# Autodesk Inventor assembly: ensemble
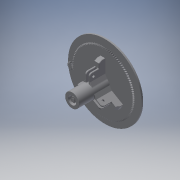
[picture p0: Inventor's stored thumbnail of the model, 180x180]
Saved by Autodesk Inventor 2019 (Build 230136000, 136)
## iProperties
Created: 2018-05-16
Part Number: ensemble
Material: Générique
Document SubType Name: Assembly
Designer: Theo
Author: Theo
## Documents named in this file (9)
- D:\dev\projects\canon-ace\ACE-T A\ensemble.iam
- D:\dev\projects\canon-ace\ACE-T A\support_principal.ipt
- D:\dev\projects\canon-ace\ACE-T A\axe_rotation_principal.ipt
- D:\dev\3d_parts\skf_6000\roulement_6000_2.iam
- D:\dev\3d_parts\emile_maurin_2201110\2201110.ipt
- D:\dev\projects\canon-ace\ACE-T A\engrenage_rotation.ipt
- D:\dev\projects\canon-ace\ACE-T A\tourelle.ipt
- D:\dev\projects\canon-ace\ACE-T A\support_serrage_tourelle.ipt
- D:\dev\projects\canon-ace\ACE-T A\engrenage_roation_1.ipt
## Components (9 placed, 8 different names)
1. support_principal:1 — Placage:1, Placage:2, Placage:4, Placage:5, Placage:6, Placage:9, Placage:10, Placage:11
2. axe_rotation_principal:1 — Placage:1, Placage:3, Placage:7, Logement:1, Placage:12, Placage:13
3. roulement_6000_2:1 [sub-assembly] — Placage:2, Placage:3, Placage:4
4. roulement_6000_2:2 [sub-assembly] — Placage:5, Placage:6, Placage:8
5. 2201110:1 — Placage:7, Placage:8
6. engrenage_rotation:1 — Placage:9, Placage:10, Placage:11
7. tourelle:1 — Logement:1, Placage:12, Placage:14, Placage:15, Placage:16
8. support_serrage_tourelle:1 — Placage:13, Placage:14, Placage:15
9. engrenage_roation_1:1 — Placage:16
## Relationships (17: Mate 16, Insert 1)
- Placage:1 [Mate]: support_principal:1 ↔ axe_rotation_principal:1
- Placage:2 [Mate]: support_principal:1 ↔ roulement_6000_2:1
- Placage:3 [Mate]: axe_rotation_principal:1 ↔ roulement_6000_2:1
- Placage:4 [Mate]: support_principal:1 ↔ roulement_6000_2:1
- Placage:5 [Mate]: support_principal:1 ↔ roulement_6000_2:2
- Placage:6 [Mate]: support_principal:1 ↔ roulement_6000_2:2
- Placage:7 [Mate]: axe_rotation_principal:1 ↔ 2201110:1
- Placage:8 [Mate]: roulement_6000_2:2 ↔ 2201110:1
- Placage:9 [Mate]: support_principal:1 ↔ engrenage_rotation:1
- Placage:10 [Mate]: support_principal:1 ↔ engrenage_rotation:1
- Placage:11 [Mate]: support_principal:1 ↔ engrenage_rotation:1
- Logement:1 [Insert]: axe_rotation_principal:1 ↔ tourelle:1
- Placage:12 [Mate]: axe_rotation_principal:1 ↔ tourelle:1
- Placage:13 [Mate]: axe_rotation_principal:1 ↔ support_serrage_tourelle:1
- Placage:14 [Mate]: tourelle:1 ↔ support_serrage_tourelle:1
- Placage:15 [Mate]: tourelle:1 ↔ support_serrage_tourelle:1
- Placage:16 [Mate]: tourelle:1 ↔ engrenage_roation_1:1
